# Autodesk Inventor assembly: A2017_T5_01
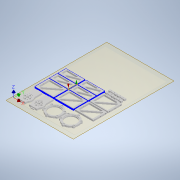
[picture p0: Inventor's stored thumbnail of the model, 180x180]
Saved by Autodesk Inventor 2020 (Build 240168000, 168)
## iProperties
Created: 2021-08-27
Part Number: A2017_T5_01
Document SubType Name: Assembly
Designer: Masato
Author: Masato
## Documents named in this file (7)
- C:\Users\marin\Documents\0111 git clone\OpenPlatform_ver3_0\cam\A2017_T5_01.iam
- C:\Users\marin\Documents\0111 git clone\OpenPlatform_ver3_0\cam\Disposable_Board.ipt
- C:\Users\marin\Documents\0111 git clone\OpenPlatform_ver3_0\LowerBody\Leg_joit\Leg_joint_yaw_frame.ipt
- C:\Users\marin\Documents\0111 git clone\OpenPlatform_ver3_0\LowerBody\Foot\Foot_root_block.ipt
- C:\Users\marin\Documents\0111 git clone\OpenPlatform_ver3_0\LowerBody\Link\FrontLink_diagonal.ipt
- C:\Users\marin\Documents\0111 git clone\OpenPlatform_ver3_0\LowerBody\Link\BackLink_diagonal.ipt
- C:\Users\marin\Documents\0111 git clone\OpenPlatform_ver3_0\UpperBody\Trunk\CrossRollerBearing\Outer_support_stand.ipt
## Components (17 placed, 6 different names)
1. Disposable_Board:1 — メイト:2, メイト:1, フラッシュ:1, フラッシュ:2, フラッシュ:3, 正接:1, 角度:1, 正接:4, フラッシュ:6, フラッシュ:8
2. Leg_joint_yaw_frame:1 — メイト:4, フラッシュ:3, 正接:1, フラッシュ:4, 正接:2, フラッシュ:5
3. Leg_joint_yaw_frame:2 — フラッシュ:4, 正接:2, フラッシュ:5, メイト:5, 正接:3, メイト:8
4. FrontLink_diagonal:4 — メイト:9, メイト:10, メイト:14, メイト:15
5. Outer_support_stand:1 — メイト:7, 角度:1, 正接:3, 正接:4
6. Outer_support_stand:3
7. FrontLink_diagonal:1 — メイト:6, フラッシュ:6, メイト:8, メイト:12
8. FrontLink_diagonal:2
9. FrontLink_diagonal:3 — メイト:10
10. BackLink_diagonal:1 — メイト:11, フラッシュ:8, メイト:12
11. BackLink_diagonal:3
12. BackLink_diagonal:4 — メイト:14
13. BackLink_diagonal:5 — メイト:16
14. Foot_root_block:1 — メイト:13, メイト:15, メイト:16
15. Foot_root_block:2
16. Foot_root_block:3
17. Foot_root_block:4
## Component patterns: (2 elements, first: Outer_support_stand:1), (3 elements, first: FrontLink_diagonal:1), (4 elements, first: BackLink_diagonal:1), (4 elements, first: Foot_root_block:1)
## Relationships (27: Mate 15, Flush 7, Tangent 4, Angle 1)
- メイト:2 [Mate]: Disposable_Board:1
- メイト:1 [Mate]: Disposable_Board:1
- フラッシュ:1 [Flush]: Disposable_Board:1
- フラッシュ:2 [Flush]: Disposable_Board:1
- メイト:4 [Mate]: Leg_joint_yaw_frame:1
- フラッシュ:3 [Flush] (3 mm): Disposable_Board:1 ↔ Leg_joint_yaw_frame:1
- 正接:1 [Tangent] (3 mm): Disposable_Board:1 ↔ Leg_joint_yaw_frame:1
- フラッシュ:4 [Flush]: Leg_joint_yaw_frame:1 ↔ Leg_joint_yaw_frame:2
- 正接:2 [Tangent] (3 mm): Leg_joint_yaw_frame:1 ↔ Leg_joint_yaw_frame:2
- フラッシュ:5 [Flush]: Leg_joint_yaw_frame:1 ↔ Leg_joint_yaw_frame:2
- メイト:5 [Mate]: Leg_joint_yaw_frame:2
- メイト:6 [Mate]: FrontLink_diagonal:1
- メイト:7 [Mate]: Outer_support_stand:1
- 角度:1 [Angle] (0 deg): Disposable_Board:1 ↔ Outer_support_stand:1
- 正接:3 [Tangent] (3 mm): Leg_joint_yaw_frame:2 ↔ Outer_support_stand:1
- 正接:4 [Tangent] (3 mm): Disposable_Board:1 ↔ Outer_support_stand:1
- フラッシュ:6 [Flush] (3 mm): Disposable_Board:1 ↔ FrontLink_diagonal:1
- メイト:8 [Mate] (3 mm): Leg_joint_yaw_frame:2 ↔ FrontLink_diagonal:1
- メイト:9 [Mate]: FrontLink_diagonal:4
- メイト:10 [Mate] (3 mm): FrontLink_diagonal:4 ↔ FrontLink_diagonal:3
- メイト:11 [Mate]: BackLink_diagonal:1
- フラッシュ:8 [Flush] (3 mm): Disposable_Board:1 ↔ BackLink_diagonal:1
- メイト:12 [Mate] (3 mm): FrontLink_diagonal:1 ↔ BackLink_diagonal:1
- メイト:13 [Mate]: Foot_root_block:1
- メイト:14 [Mate] (5 mm): FrontLink_diagonal:4 ↔ BackLink_diagonal:4
- メイト:15 [Mate] (3 mm): FrontLink_diagonal:4 ↔ Foot_root_block:1
- メイト:16 [Mate] (5 mm): BackLink_diagonal:5 ↔ Foot_root_block:1
